# Autodesk Inventor assembly: Slider with leds
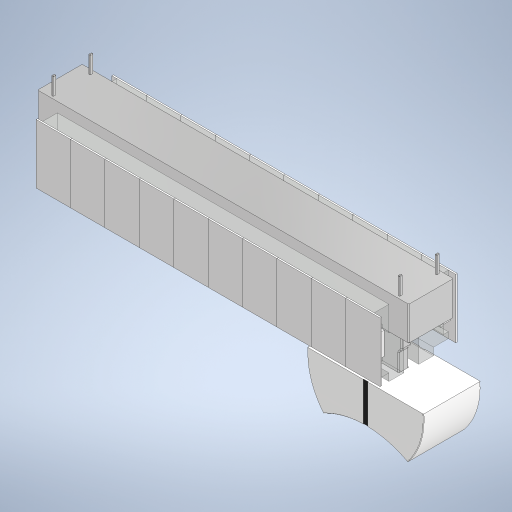
[picture p0: Inventor's stored thumbnail of the model, 512x512]
Saved by Autodesk Inventor 2023 (Build 270158000, 158)
## iProperties
Created: 2024-03-26
Part Number: Slider with leds
Document SubType Name: Assembly
Designer: noname
Author: noname
## Documents named in this file (4)
- C:\Users\noname\Documents\GitHub\AudMix\3dModels\Slider with leds.iam
- C:\Users\noname\Documents\GitHub\AudMix\3dModels\Slider\SliderAssembly.iam
- C:\Users\noname\Documents\GitHub\AudMix\3dModels\LedStrip\144x10.iam
- C:\Users\noname\Documents\GitHub\AudMix\3dModels\Diffuser.ipt
## Components (5 placed, 3 different names)
1. SliderAssembly:1 [sub-assembly] — Mate:1, Mate:2, Mate:3, Mate:4, Flush:1
2. 144x10:1 [sub-assembly] — Mate:6, Flush:5, Flush:6, Symmetry:1
3. 144x10:2 [sub-assembly] — Mate:5, Flush:3, Flush:4, Flush:5, Symmetry:1
4. Diffuser:1 — Mate:2, Mate:4, Flush:2, Mate:6, Flush:6, Symmetry:2
5. Diffuser:2 — Mate:1, Mate:3, Flush:1, Flush:2, Mate:5, Flush:3, Flush:4, Symmetry:2
## Relationships (14: Mate 6, Flush 6, Symmetry 2)
- Mate:1: SliderAssembly:1 ↔ Diffuser:2
- Mate:2: SliderAssembly:1 ↔ Diffuser:1
- Mate:3: SliderAssembly:1 ↔ Diffuser:2
- Mate:4: SliderAssembly:1 ↔ Diffuser:1
- Flush:1 (4 mm): SliderAssembly:1 ↔ Diffuser:2
- Flush:2: Diffuser:1 ↔ Diffuser:2
- Mate:5: 144x10:2 ↔ Diffuser:2
- Flush:3: 144x10:2 ↔ Diffuser:2
- Flush:4 (-1 mm): 144x10:2 ↔ Diffuser:2
- Mate:6: 144x10:1 ↔ Diffuser:1
- Flush:5: 144x10:1 ↔ 144x10:2
- Flush:6: 144x10:1 ↔ Diffuser:1
- Symmetry:1: 144x10:1 ↔ 144x10:2
- Symmetry:2: Diffuser:1 ↔ Diffuser:2
